# Autodesk Inventor assembly: PaddleCollection2.1.ipt
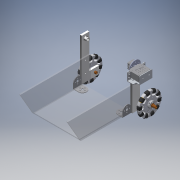
[picture p0: Inventor's stored thumbnail of the model, 180x180]
Saved by Autodesk Inventor 2019 (Build 230136000, 136)
## iProperties
Created: 2018-10-20
Part Number: PaddleCollection2.1.ipt
Document SubType Name: Assembly
Designer: User
Author: User
## Documents named in this file (17)
- C:\Robotics\CAD\2018-19_CAD\Collection\PaddleCollection2.1.ipt.iam
- C:\Robotics\CAD\2018-19_CAD\Collection\PaddleCollection2.1AxleSupport.ipt
- C:\Robotics\CAD\2018-19_CAD\Collection\PaddleCollection2.1Casing.ipt
- C:\Robotics\CAD\2018-19_CAD\Collection\PaddleCollectionFloor.ipt
- C:\Robotics\CAD\COTSParts\Tetrix\Tetrix Wheel 3 in omni.ipt
- C:\Robotics\CAD\COTSParts\Tetrix\Bronze bushing.ipt
- C:\Robotics\CAD\COTSParts\Tetrix\Tetrix shaft collar.ipt
- C:\Robotics\CAD\COTSParts\Tetrix\Tetrix Hub - axle.ipt
- C:\Robotics\CAD\COTSParts\Rev\REV-41-1097SmartServo.ipt
- C:\Robotics\CAD\COTSParts\Tetrix\39060_txm-standard servo bracket.ipt
- C:\Robotics\CAD\COTSParts\Tetrix\Tetrix bracket - angle.ipt
- C:\Robotics\CAD\2018-19_CAD\Collection\PaddleCollection2.1ServoSupport.ipt
- C:\Robotics\CAD\COTSParts\Bearings - AndyMark\Bearing 250 ID 500 OD flanged.ipt
- C:\Robotics\CAD\COTSParts\Actobotics\Collar.ipt
- C:\Robotics\CAD\COTSParts\Rev\REV-41-1363ServoHorn.ipt
- C:\Robotics\CAD\COTSParts\Actobotics\545 parts\545456PatternAdapter.77in.625in.ipt
- C:\Robotics\CAD\COTSParts\Actobotics\545 parts\545548SetScrewHub.77inPattern.ipt
## Components (25 placed, 16 different names)
1. PaddleCollection2.1AxleSupport:1 — Mate:1, Mate:2, Flush:1, Insert:1, Insert:15, Mate:14
2. PaddleCollection2.1Casing:1 — Flush:3, Mate:5, Mate:6, Mate:1, Mate:13
3. PaddleCollection2.1Casing:2 — Mate:3, Mate:4, Flush:2, Flush:4, Mate:8, Flush:5, Mate:10
4. PaddleCollectionFloor:1 — Mate:2, Flush:1, Mate:3, Mate:4, Flush:2, Flush:3, Mate:5, Mate:6, Mate:9, Mate:12
5. Tetrix Wheel 3 in omni:1 — Insert:3, Insert:4
6. Bronze bushing:1 — Insert:1, Insert:2
7. Bronze bushing:2 — Insert:5
8. Tetrix shaft collar:1 — Insert:2, Insert:3
9. Tetrix Hub - axle:1 — Insert:4, Insert:5
10. REV-41-1097SmartServo:1 — Insert:6, Angle:1, Insert:17
11. 39060_txm-standard servo bracket:1 — Insert:6, Angle:1, Insert:7, Insert:8
12. Tetrix bracket - angle:1 — Insert:7, Insert:8, Insert:9, Angle:2
13. PaddleCollection2.1ServoSupport:1 — Flush:4, Mate:8, Flush:5, Insert:9, Angle:2, Insert:10, Mate:11
14. Bronze bushing:3 — Insert:14
15. Tetrix Wheel 3 in omni:2 — Insert:12, Insert:13
16. Tetrix shaft collar:2 — Insert:11, Insert:12
17. Tetrix Hub - axle:2 — Insert:13, Insert:14
18. Bronze bushing:4 — Insert:10, Insert:11
19. Bearing 250 ID 500 OD flanged:1 — Insert:15, Insert:16
20. Collar:1 — Insert:16
21. Tetrix bracket - angle:2 — Mate:9, Mate:10, Mate:11
22. Tetrix bracket - angle:3 — Mate:12, Mate:13, Mate:14
23. REV-41-1363ServoHorn:1 — Insert:17, Insert:18
24. 545456PatternAdapter.77in.625in:1 — Insert:18, Insert:19
25. 545548SetScrewHub.77inPattern:1 — Insert:19
## Relationships (39: Insert 19, Mate 13, Flush 5, Angle 2)
- Mate:1: PaddleCollection2.1AxleSupport:1 ↔ PaddleCollection2.1Casing:1
- Mate:2: PaddleCollection2.1AxleSupport:1 ↔ PaddleCollectionFloor:1
- Flush:1: PaddleCollection2.1AxleSupport:1 ↔ PaddleCollectionFloor:1
- Mate:3: PaddleCollection2.1Casing:2 ↔ PaddleCollectionFloor:1
- Mate:4: PaddleCollection2.1Casing:2 ↔ PaddleCollectionFloor:1
- Flush:2: PaddleCollection2.1Casing:2 ↔ PaddleCollectionFloor:1
- Flush:3: PaddleCollection2.1Casing:1 ↔ PaddleCollectionFloor:1
- Mate:5: PaddleCollection2.1Casing:1 ↔ PaddleCollectionFloor:1
- Mate:6: PaddleCollection2.1Casing:1 ↔ PaddleCollectionFloor:1
- Insert:1: PaddleCollection2.1AxleSupport:1 ↔ Bronze bushing:1
- Insert:2: Bronze bushing:1 ↔ Tetrix shaft collar:1
- Insert:3: Tetrix Wheel 3 in omni:1 ↔ Tetrix shaft collar:1
- Insert:4: Tetrix Wheel 3 in omni:1 ↔ Tetrix Hub - axle:1
- Insert:5: Bronze bushing:2 ↔ Tetrix Hub - axle:1
- Insert:6: REV-41-1097SmartServo:1 ↔ 39060_txm-standard servo bracket:1
- Angle:1 (0 deg): REV-41-1097SmartServo:1 ↔ 39060_txm-standard servo bracket:1
- Insert:7: 39060_txm-standard servo bracket:1 ↔ Tetrix bracket - angle:1
- Insert:8: 39060_txm-standard servo bracket:1 ↔ Tetrix bracket - angle:1
- Flush:4: PaddleCollection2.1Casing:2 ↔ PaddleCollection2.1ServoSupport:1
- Mate:8: PaddleCollection2.1Casing:2 ↔ PaddleCollection2.1ServoSupport:1
- Flush:5: PaddleCollection2.1Casing:2 ↔ PaddleCollection2.1ServoSupport:1
- Insert:9: Tetrix bracket - angle:1 ↔ PaddleCollection2.1ServoSupport:1
- Angle:2 (0 deg): Tetrix bracket - angle:1 ↔ PaddleCollection2.1ServoSupport:1
- Insert:10: PaddleCollection2.1ServoSupport:1 ↔ Bronze bushing:4
- Insert:11: Tetrix shaft collar:2 ↔ Bronze bushing:4
- Insert:12: Tetrix Wheel 3 in omni:2 ↔ Tetrix shaft collar:2
- Insert:13: Tetrix Wheel 3 in omni:2 ↔ Tetrix Hub - axle:2
- Insert:14: Bronze bushing:3 ↔ Tetrix Hub - axle:2
- Insert:15: PaddleCollection2.1AxleSupport:1 ↔ Bearing 250 ID 500 OD flanged:1
- Insert:16: Bearing 250 ID 500 OD flanged:1 ↔ Collar:1
- Mate:9: PaddleCollectionFloor:1 ↔ Tetrix bracket - angle:2
- Mate:10: PaddleCollection2.1Casing:2 ↔ Tetrix bracket - angle:2
- Mate:11: PaddleCollection2.1ServoSupport:1 ↔ Tetrix bracket - angle:2
- Mate:12: PaddleCollectionFloor:1 ↔ Tetrix bracket - angle:3
- Mate:13: PaddleCollection2.1Casing:1 ↔ Tetrix bracket - angle:3
- Mate:14: PaddleCollection2.1AxleSupport:1 ↔ Tetrix bracket - angle:3
- Insert:17: REV-41-1097SmartServo:1 ↔ REV-41-1363ServoHorn:1
- Insert:18: REV-41-1363ServoHorn:1 ↔ 545456PatternAdapter.77in.625in:1
- Insert:19: 545456PatternAdapter.77in.625in:1 ↔ 545548SetScrewHub.77inPattern:1
